# Autodesk Inventor assembly: ロボット回転
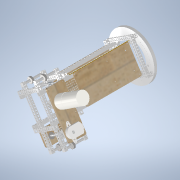
[picture p0: Inventor's stored thumbnail of the model, 180x180]
Saved by Autodesk Inventor 2020.3 (Build 243373000, 373)
## iProperties
Created: 2020-07-04
Part Number: ロボット回転
Document SubType Name: Assembly
Designer: totot
Mass: 811.068 g
Surface Area: 2821.31 cm^2
Volume: 358.782 cm^3
Density: 2.26062 g/cm^3
Author: totot
## Documents named in this file (20)
- D:\mysvn\ロボコン\キャチロボ\キャチロボ設計図\ロボット\ロボット回転\ロボット回転.iam
- D:\mysvn\ロボコン\キャチロボ\キャチロボ設計図\ロボット\共有パーツ\turntable1.ipt
- D:\mysvn\ロボコン\キャチロボ\キャチロボ設計図\ロボット\共有パーツ\turntable2.ipt
- D:\mysvn\ロボコン\キャチロボ\キャチロボ設計図\ロボット\ロボット回転\ロボット回転9ｘ9_1.ipt
- D:\mysvn\ロボコン\キャチロボ\キャチロボ設計図\ロボット\ロボット回転\ロボット回転9x9_2.ipt
- D:\mysvn\ロボコン\キャチロボ\キャチロボ設計図\ロボット\ロボット回転\ロボット回転9x9_3.ipt
- D:\mysvn\ロボコン\キャチロボ\キャチロボ設計図\ロボット\ロボット回転\ロボット回転t5.5.ipt
- D:\mysvn\ロボコン\キャチロボ\キャチロボ設計図\ロボット\共有パーツ\RS_540.ipt
- D:\mysvn\ロボコン\キャチロボ\キャチロボ設計図\ロボット\共有パーツ\PS1-20_On.ipt
- D:\mysvn\ロボコン\キャチロボ\キャチロボ設計図\ロボット\ロボット回転\ロボット回転_ベアリングシャフト縦.ipt
- D:\mysvn\ロボコン\キャチロボ\キャチロボ設計図\ロボット\ロボット回転\ロボット回転_ベアリングシャフト横.ipt
- D:\mysvn\ロボコン\キャチロボ\キャチロボ設計図\ロボット\ロボット回転\ロボット回転9x9_4.ipt
- D:\mysvn\ロボコン\キャチロボ\キャチロボ設計図\ロボット\ハンド\ハンド_ベアリング_4-8.ipt
- D:\mysvn\ロボコン\キャチロボ\キャチロボ設計図\ロボット\共有パーツ\ベアリング_6-17.ipt
- D:\mysvn\ロボコン\キャチロボ\キャチロボ設計図\ロボット\ロボット回転\ロボット回転_回路ボード1.ipt
- D:\mysvn\ロボコン\キャチロボ\キャチロボ設計図\ロボット\ロボット回転\ロボット回転_回路ボード1_CPY.ipt
- D:\mysvn\ロボコン\キャチロボ\キャチロボ設計図\ロボット\共有パーツ\AMT102-Vwide.ipt
- D:\mysvn\ロボコン\キャチロボ\キャチロボ設計図\ロボット\ロボット回転\ロボット回転t5.5_2.ipt
- D:\mysvn\ロボコン\キャチロボ\キャチロボ設計図\ロボット\ロボット回転\ロボット回転_エンコーダシャフト.ipt
- D:\mysvn\ロボコン\キャチロボ\キャチロボ設計図\ロボット\共有パーツ\F606ZZ\F606ZZ.iam
## Components (42 placed, 19 different names)
1. turntable1:1 — 正接:1, フラッシュ:1
2. turntable2:1 — 正接:1, フラッシュ:1, 挿入:3, 挿入:4, 挿入:9, 挿入:11
3. ロボット回転9ｘ9_1:1 — 挿入:3, 挿入:4, 挿入:6, 挿入:8, 挿入:64, 挿入:73
4. ロボット回転9ｘ9_1:2 — 挿入:9, 挿入:10, 挿入:11, 挿入:12, 挿入:58, 挿入:60
5. ロボット回転9ｘ9_1:3 — 挿入:8, 挿入:10
6. ロボット回転9ｘ9_1:4 — 挿入:6, 挿入:12, 挿入:59, 挿入:63
7. ロボット回転_ベアリングシャフト縦:1 — 挿入:24, 挿入:29, 挿入:96
8. ロボット回転9x9_2:1 — 挿入:55, 挿入:56, 挿入:57, 挿入:58, 挿入:59, 挿入:92, 挿入:105, フラッシュ:2, メイト:1
9. ロボット回転9x9_2:2 — 挿入:60, 挿入:61, 挿入:69, 挿入:70, 挿入:82, 挿入:85, 挿入:90, 挿入:102, 挿入:103, 挿入:106
10. ロボット回転9x9_3:1 — 挿入:35, 挿入:36, 挿入:70, 挿入:71, 挿入:93
11. ロボット回転t5.5:1 — 挿入:82, 挿入:83, 挿入:84, 挿入:85, 挿入:86, 挿入:87, 挿入:98, 挿入:99
12. RS_540:1 — 挿入:98, 挿入:99, 挿入:104
13. PS1-20_On:1 — 挿入:104
14. ロボット回転9x9_2:3 — 挿入:67, 挿入:71, 挿入:72, 挿入:73, 挿入:74, 挿入:83, 挿入:84, 挿入:100, 挿入:101, 挿入:109
15. ロボット回転9x9_2:4 — 挿入:63, 挿入:64, 挿入:65, 挿入:77, 挿入:110
16. ロボット回転9x9_3:2 — 挿入:29, 挿入:31, 挿入:55, 挿入:66, 挿入:78, 挿入:81, 挿入:91
17. ロボット回転9x9_3:3 — 挿入:24, 挿入:30, 挿入:56, 挿入:76, 挿入:79, 挿入:80
18. ロボット回転9x9_3:4 — 挿入:34, 挿入:37, 挿入:68, 挿入:69, 挿入:72, 挿入:75
19. ロボット回転_ベアリングシャフト縦:2 — 挿入:34, 挿入:35, 挿入:97
20. ロボット回転_ベアリングシャフト縦:3 — 挿入:36, 挿入:37, 挿入:94
21. ロボット回転_ベアリングシャフト縦:4 — 挿入:30, 挿入:31, 挿入:95
22. ロボット回転_ベアリングシャフト横:1 — 挿入:105, 挿入:106, 挿入:107, 挿入:108
23. ロボット回転_ベアリングシャフト横:2 — 挿入:109, 挿入:110, 挿入:111, 挿入:112
24. ロボット回転9x9_4:1 — 挿入:90, 挿入:91, 挿入:92, 挿入:93
25. ロボット回転9x9_4:2 — 挿入:65, 挿入:66, 挿入:67
26. ハンド_ベアリング_4-8:1 — 挿入:112
27. ハンド_ベアリング_4-8:2 — 挿入:111
28. ハンド_ベアリング_4-8:3 — 挿入:107
29. ハンド_ベアリング_4-8:4 — 挿入:108
30. ベアリング_6-17:1 — 挿入:94
31. ベアリング_6-17:2 — 挿入:97
32. ベアリング_6-17:6 — 挿入:95
33. ベアリング_6-17:7 — 挿入:96
34. ロボット回転_回路ボード1:1 — フラッシュ:2, メイト:1, フラッシュ:3
35. ロボット回転_回路ボード1_CPY:1 — 挿入:100, 挿入:101, 挿入:102, 挿入:103, フラッシュ:3
36. AMT102-Vwide:1 — 挿入:86, 挿入:87, 挿入:88
37. PS1-20_On:2 — 挿入:89
38. ロボット回転t5.5_2:1 — 挿入:32, 挿入:78, 挿入:79, 挿入:80, 挿入:81
39. ロボット回転_エンコーダシャフト:1 — 挿入:88, 挿入:89
40. F606ZZ:1 [sub-assembly] — 挿入:32
41. ロボット回転9x9_4:3 — 挿入:57, 挿入:61, 挿入:68
42. ロボット回転9x9_4:4 — 挿入:74, 挿入:75, 挿入:76, 挿入:77
## Relationships (79: Insert 74, Flush 3, Tangent 1, Mate 1)
- 正接:1 [Tangent]: turntable1:1 ↔ turntable2:1
- フラッシュ:1 [Flush]: turntable1:1 ↔ turntable2:1
- 挿入:3 [Insert]: turntable2:1 ↔ ロボット回転9ｘ9_1:1
- 挿入:4 [Insert]: turntable2:1 ↔ ロボット回転9ｘ9_1:1
- 挿入:6 [Insert]: ロボット回転9ｘ9_1:1 ↔ ロボット回転9ｘ9_1:4
- 挿入:8 [Insert]: ロボット回転9ｘ9_1:1 ↔ ロボット回転9ｘ9_1:3
- 挿入:9 [Insert]: turntable2:1 ↔ ロボット回転9ｘ9_1:2
- 挿入:10 [Insert]: ロボット回転9ｘ9_1:2 ↔ ロボット回転9ｘ9_1:3
- 挿入:11 [Insert]: turntable2:1 ↔ ロボット回転9ｘ9_1:2
- 挿入:12 [Insert]: ロボット回転9ｘ9_1:2 ↔ ロボット回転9ｘ9_1:4
- 挿入:24 [Insert]: ロボット回転_ベアリングシャフト縦:1 ↔ ロボット回転9x9_3:3
- 挿入:29 [Insert]: ロボット回転_ベアリングシャフト縦:1 ↔ ロボット回転9x9_3:2
- 挿入:30 [Insert]: ロボット回転9x9_3:3 ↔ ロボット回転_ベアリングシャフト縦:4
- 挿入:31 [Insert]: ロボット回転9x9_3:2 ↔ ロボット回転_ベアリングシャフト縦:4
- 挿入:32 [Insert]: ロボット回転t5.5_2:1 ↔ F606ZZ:1
- 挿入:34 [Insert]: ロボット回転9x9_3:4 ↔ ロボット回転_ベアリングシャフト縦:2
- 挿入:35 [Insert]: ロボット回転9x9_3:1 ↔ ロボット回転_ベアリングシャフト縦:2
- 挿入:36 [Insert]: ロボット回転9x9_3:1 ↔ ロボット回転_ベアリングシャフト縦:3
- 挿入:37 [Insert]: ロボット回転9x9_3:4 ↔ ロボット回転_ベアリングシャフト縦:3
- 挿入:55 [Insert]: ロボット回転9x9_2:1 ↔ ロボット回転9x9_3:2
- 挿入:56 [Insert]: ロボット回転9x9_2:1 ↔ ロボット回転9x9_3:3
- 挿入:57 [Insert]: ロボット回転9x9_2:1 ↔ ロボット回転9x9_4:3
- 挿入:58 [Insert]: ロボット回転9ｘ9_1:2 ↔ ロボット回転9x9_2:1
- 挿入:59 [Insert]: ロボット回転9ｘ9_1:4 ↔ ロボット回転9x9_2:1
- 挿入:60 [Insert]: ロボット回転9ｘ9_1:2 ↔ ロボット回転9x9_2:2
- 挿入:61 [Insert]: ロボット回転9x9_2:2 ↔ ロボット回転9x9_4:3
- 挿入:63 [Insert]: ロボット回転9ｘ9_1:4 ↔ ロボット回転9x9_2:4
- 挿入:64 [Insert]: ロボット回転9ｘ9_1:1 ↔ ロボット回転9x9_2:4
- 挿入:65 [Insert]: ロボット回転9x9_2:4 ↔ ロボット回転9x9_4:2
- 挿入:66 [Insert]: ロボット回転9x9_3:2 ↔ ロボット回転9x9_4:2
- 挿入:67 [Insert]: ロボット回転9x9_2:3 ↔ ロボット回転9x9_4:2
- 挿入:68 [Insert]: ロボット回転9x9_3:4 ↔ ロボット回転9x9_4:3
- 挿入:69 [Insert]: ロボット回転9x9_2:2 ↔ ロボット回転9x9_3:4
- 挿入:70 [Insert]: ロボット回転9x9_2:2 ↔ ロボット回転9x9_3:1
- 挿入:71 [Insert]: ロボット回転9x9_3:1 ↔ ロボット回転9x9_2:3
- 挿入:72 [Insert]: ロボット回転9x9_2:3 ↔ ロボット回転9x9_3:4
- 挿入:73 [Insert]: ロボット回転9ｘ9_1:1 ↔ ロボット回転9x9_2:3
- 挿入:74 [Insert]: ロボット回転9x9_2:3 ↔ ロボット回転9x9_4:4
- 挿入:75 [Insert]: ロボット回転9x9_3:4 ↔ ロボット回転9x9_4:4
- 挿入:76 [Insert]: ロボット回転9x9_3:3 ↔ ロボット回転9x9_4:4
- 挿入:77 [Insert]: ロボット回転9x9_2:4 ↔ ロボット回転9x9_4:4
- 挿入:78 [Insert]: ロボット回転9x9_3:2 ↔ ロボット回転t5.5_2:1
- 挿入:79 [Insert]: ロボット回転9x9_3:3 ↔ ロボット回転t5.5_2:1
- 挿入:80 [Insert]: ロボット回転9x9_3:3 ↔ ロボット回転t5.5_2:1
- 挿入:81 [Insert]: ロボット回転9x9_3:2 ↔ ロボット回転t5.5_2:1
- 挿入:82 [Insert]: ロボット回転9x9_2:2 ↔ ロボット回転t5.5:1
- 挿入:83 [Insert]: ロボット回転t5.5:1 ↔ ロボット回転9x9_2:3
- 挿入:84 [Insert]: ロボット回転t5.5:1 ↔ ロボット回転9x9_2:3
- 挿入:85 [Insert]: ロボット回転9x9_2:2 ↔ ロボット回転t5.5:1
- 挿入:86 [Insert]: ロボット回転t5.5:1 ↔ AMT102-Vwide:1
- 挿入:87 [Insert]: ロボット回転t5.5:1 ↔ AMT102-Vwide:1
- 挿入:88 [Insert]: AMT102-Vwide:1 ↔ ロボット回転_エンコーダシャフト:1
- 挿入:89 [Insert] (-60 mm): PS1-20_On:2 ↔ ロボット回転_エンコーダシャフト:1
- 挿入:90 [Insert]: ロボット回転9x9_2:2 ↔ ロボット回転9x9_4:1
- 挿入:91 [Insert]: ロボット回転9x9_3:2 ↔ ロボット回転9x9_4:1
- 挿入:92 [Insert]: ロボット回転9x9_2:1 ↔ ロボット回転9x9_4:1
- 挿入:93 [Insert]: ロボット回転9x9_3:1 ↔ ロボット回転9x9_4:1
- 挿入:94 [Insert] (-30 mm): ロボット回転_ベアリングシャフト縦:3 ↔ ベアリング_6-17:1
- 挿入:95 [Insert] (-30 mm): ロボット回転_ベアリングシャフト縦:4 ↔ ベアリング_6-17:6
- 挿入:96 [Insert] (-30 mm): ロボット回転_ベアリングシャフト縦:1 ↔ ベアリング_6-17:7
- 挿入:97 [Insert] (-30 mm): ロボット回転_ベアリングシャフト縦:2 ↔ ベアリング_6-17:2
- 挿入:98 [Insert]: ロボット回転t5.5:1 ↔ RS_540:1
- 挿入:99 [Insert]: ロボット回転t5.5:1 ↔ RS_540:1
- 挿入:100 [Insert]: ロボット回転9x9_2:3 ↔ ロボット回転_回路ボード1_CPY:1
- 挿入:101 [Insert]: ロボット回転9x9_2:3 ↔ ロボット回転_回路ボード1_CPY:1
- 挿入:102 [Insert]: ロボット回転9x9_2:2 ↔ ロボット回転_回路ボード1_CPY:1
- 挿入:103 [Insert]: ロボット回転9x9_2:2 ↔ ロボット回転_回路ボード1_CPY:1
- 挿入:104 [Insert] (5 mm): RS_540:1 ↔ PS1-20_On:1
- 挿入:105 [Insert]: ロボット回転9x9_2:1 ↔ ロボット回転_ベアリングシャフト横:1
- 挿入:106 [Insert]: ロボット回転9x9_2:2 ↔ ロボット回転_ベアリングシャフト横:1
- 挿入:107 [Insert] (-30 mm): ロボット回転_ベアリングシャフト横:1 ↔ ハンド_ベアリング_4-8:3
- 挿入:108 [Insert] (-25 mm): ロボット回転_ベアリングシャフト横:1 ↔ ハンド_ベアリング_4-8:4
- 挿入:109 [Insert]: ロボット回転9x9_2:3 ↔ ロボット回転_ベアリングシャフト横:2
- 挿入:110 [Insert]: ロボット回転9x9_2:4 ↔ ロボット回転_ベアリングシャフト横:2
- 挿入:111 [Insert] (-30 mm): ロボット回転_ベアリングシャフト横:2 ↔ ハンド_ベアリング_4-8:2
- 挿入:112 [Insert] (-25 mm): ロボット回転_ベアリングシャフト横:2 ↔ ハンド_ベアリング_4-8:1
- フラッシュ:2 [Flush]: ロボット回転9x9_2:1 ↔ ロボット回転_回路ボード1:1
- メイト:1 [Mate]: ロボット回転9x9_2:1 ↔ ロボット回転_回路ボード1:1
- フラッシュ:3 [Flush]: ロボット回転_回路ボード1:1 ↔ ロボット回転_回路ボード1_CPY:1
